# Autodesk Inventor assembly: PowerPlantShaftAssembely
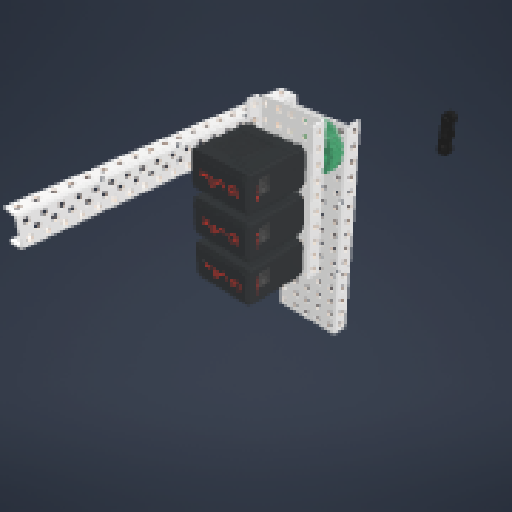
[picture p0: Inventor's stored thumbnail of the model, 512x512]
Saved by Autodesk Inventor 2023 (Build 270158000, 158)
## iProperties
Created: 2023-05-01
Part Number: PowerPlantShaftAssembely
Document SubType Name: Assembly
Designer: alex
Author: alex
## Documents named in this file (9)
- C:\Users\alex\Documents\GitHub\4067X-Over-Under-CAD\PowerPlantShaftAssembely.iam
- C:\Users\alex\Documents\GitHub\4067x_2023-24_cad\VEX-CAD-Inventor\Motion\Gears\HS Gear\HS 36T Gear, Square Old.ipt
- C:\Users\alex\Documents\GitHub\4067x_2023-24_cad\VEX-CAD-Inventor\Motion\Spacers\Spacer Nylon .375 OD\NSpacer .375 OD x .125.ipt
- C:\Users\alex\Documents\GitHub\4067x_2023-24_cad\VEX-CAD-Inventor\Motion\Spacers\Spacer Nylon .375 OD.ipt
- C:\Users\alex\Documents\GitHub\4067x_2023-24_cad\VEX-CAD-Inventor\Motion\Shaft LS\Shaft Collar ipts\Shaft Collar Set Screw.ipt
- C:\Users\alex\Documents\GitHub\4067x_2023-24_cad\VEX-CAD-Inventor\Motion\Spacers\Washer Steel\SWasher .375 OD x .015625.ipt
- C:\Users\alex\Documents\GitHub\4067x_2023-24_cad\VEX-CAD-Inventor\Motion\Spacers\Washer Steel.ipt
- C:\Users\alex\Documents\GitHub\4067x_2023-24_cad\VEX-CAD-Inventor\Motion\Shaft LS\Shaft LS\Shaft LS 2.0.ipt
- C:\Users\alex\Documents\GitHub\4067x_2023-24_cad\VEX-CAD-Inventor\Motion\Shaft LS\Shaft LS.ipt
## Components (5 placed, 5 different names)
1. HS 36T Gear, Square Old:1 — Insert:6, Insert:17, Mate:5, Mate:6
2. Shaft Collar Set Screw:1 — Insert:6, Insert:16
3. SWasher .375 OD x .015625:1 — Insert:16, Flush:1
4. NSpacer .375 OD x .125:1 — Insert:17
5. Shaft LS 2.0:1 — Mate:5, Mate:6, Flush:1
## Relationships (6: Insert 3, Mate 2, Flush 1)
- Insert:6: HS 36T Gear, Square Old:1 ↔ Shaft Collar Set Screw:1
- Insert:16: Shaft Collar Set Screw:1 ↔ SWasher .375 OD x .015625:1
- Insert:17: HS 36T Gear, Square Old:1 ↔ NSpacer .375 OD x .125:1
- Mate:5: HS 36T Gear, Square Old:1 ↔ Shaft LS 2.0:1
- Mate:6: HS 36T Gear, Square Old:1 ↔ Shaft LS 2.0:1
- Flush:1 (-23.9875 mm): SWasher .375 OD x .015625:1 ↔ Shaft LS 2.0:1
